# Autodesk Inventor assembly: injector assembly
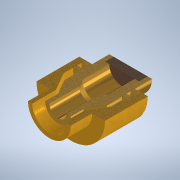
[picture p0: Inventor's stored thumbnail of the model, 180x180]
Saved by Autodesk Inventor 2021 (Build 250183000, 183)
## iProperties
Created: 2021-07-21
Part Number: injector assembly
Document SubType Name: Assembly
Designer: samlo
Author: samlo
## Documents named in this file (4)
- C:\Users\samlo\OneDrive\Documents\injector assembly.iam
- C:\Users\samlo\OneDrive\Documents\bottom injector.ipt
- C:\Users\samlo\OneDrive\Documents\inner element.ipt
- C:\Users\samlo\OneDrive\Documents\cap injector.ipt
## Components (3 placed, 3 different names)
1. bottom injector:1 — Rigid:1
2. inner element:1 — Rigid:1, Rigid:2
3. cap injector:1 — Rigid:2
## Relationships (2: WeldJoint 2)
- Rigid:1 [WeldJoint]: bottom injector:1 ↔ inner element:1
- Rigid:2 [WeldJoint]: inner element:1 ↔ cap injector:1
